# Autodesk Inventor assembly: MHPUS306-50-25-A
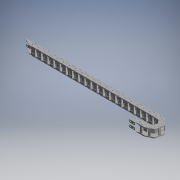
[picture p0: Inventor's stored thumbnail of the model, 180x180]
Saved by Autodesk Inventor 2017.3 (Build 213256000, 256)
## iProperties
Category: PARTsolutions
Company: MISUMI
Part Number: MHPUS306-50-25-A
Catalog Web Link: www.cadenas.de
Description: MHPUS-Cable Carriers - Flap Open-Close Type
Vendor: MISUMI
Document SubType Name: Assembly
Designer: partserver
Manufacturer: MISUMI
Mass: 772.343 g
Surface Area: 4615.68 cm^2
Volume: 772.343 cm^3
Density: 1 g/cm^3
Title: MHPUS306-50-25-A
Author: Cadenas PARTsolutions
Comments: Cable Carriers - Flap Open-Close Type
PSOL_IDENT_0: {$CADENAS_DATA\23d-libs\misumi\metric\07_slide_rails\mhpus_asmtab.prj},191 {VTYP=3D},{STYP=ASSTAB},{
PSOL_IDENT_1: NB=MHPUS306-50-25-A},{LINA=MHPUS306-50-25-A},{NN=MHPUS},{DATE=30.06.2021 12:53:59},{GEOMDATE=16.03.2
PSOL_IDENT_2: 015},{VERSION=},{LINEID=90},{WBVAR=BR,NOL,AD},{WBNUMERIC=BR,NOL}  {NB=MHPUS306-50-25-A},{LINA=MHPUS3
PSOL_IDENT_3: 06-50-25-A},{KT=DUMMY},{PN=MHPUS306-50-25-A},{MATB=Nylon 6 + Glass 20 percent},{OT=-10~80},{MATFB=Lo
PSOL_IDENT_4: w Carbon SteelC},{STFB=Trivalent Bright Chromate Plating},{NO=306},{BR=50},{BRA=50,100},{NOL=25},{NO
PSOL_IDENT_5: LALG=[6-38/1]},{AD=A},{ADALG= 'A', 'Outer circumference', 'B', 'Inner circumference' },{A=24.0},{B=3
PSOL_IDENT_6: 4},{C=44},{W=60},{P=45},{LL=60},{F=40},{T=24},{J=20},{N=7.0},{P1F=35.6},{P2F=55.6},{P1FX=32},{P2FX=5
PSOL_IDENT_7: 2},{H=134},{H1=100},{HF=160},{K=257.0},{WT=0.64},{ANGLE=53.48737},{ANGLE2=0.00000},{ANGLE3=90.00000}
PSOL_IDENT_8: ,{GAMA=27.52031},{GAMA2=0.00000},{GAMA3=nan},{BETA=45.50496},{BETA2=0.00000},{BETA3=0.00000},{X0=17.
PSOL_IDENT_9: 00000},{Y0=0.00000},{X1=-28.00000},{Y1=0.00000},{X2=-54.77500},{Y2=36.16766},{X3=-41.63725},{Y3=79.2
PSOL_IDENT_10: 0717},{X4=0.77167},{Y4=94.25653},{X5=38.10054},{Y5=69.12576},{X6=0.00000},{Y6=0.00000},{X7=0.00000},
PSOL_IDENT_11: {Y7=100.00000},{X8=45.00000},{Y8=100.00000},{R1=11.5},{R2=8.0},{R3=2.000},{L1=3.500},{L2=19.6905},{L
PSOL_IDENT_12: 3=3.700},{CL1=-26.743683950},{CL2=-53.487367900},{CL3=-53.487367900},{CL4=-42.613450190},{CL5=-3.668
PSOL_IDENT_13: 130050},{CL6=0.000000000},{CL7=0.000000000},{CL8=0.000000000},{CL9=0.000000000},{CL10=0.000000000},{
PSOL_IDENT_14: CL11=0.000000000},{CL12=0.000000000},{TILT=0},{PPATH=mhpus_asmtpl.prj}
NB: MHPUS306-50-25-A
NN: MHPUS
NT: Cable Carriers - Flap Open-Close Type
NBSYN: $PN.
LINA: MHPUS306-50-25-A
CATALOG: Misumi
PN: MHPUS306-50-25-A
MATB: Nylon 6 + Glass 20 percent
OT: -10~80
MATFB: Low Carbon SteelC
STFB: Trivalent Bright Chromate Plating
NO: 306
BR: 50
NOL: 25
AD: Outer circumference
A: 24
B: 34
C: 44
W: 60
P: 45
LL: 60
F: 40
T: 24
J: 20
N: 7
P1F: 35.6
P2F: 55.6
P1FX: 32
P2FX: 52
H: 134
H1: 100
HF: 160
K: 257
WT: 0.64
SUPPLIER: MISUMI
ARTICLENO: MHPUS306-50-25-A
BOMINFO: MHPUS306-50-25-A
CREATOR: CADENAS GmbH
## Documents named in this file (6)
- e:\temp\worker_7\temp\exporttempdir_952_134_K7orS\format_0\MHPUS306-50-25-A.iam
- e:\temp\worker_7\temp\exporttempdir_952_134_K7orS\format_0\MHPUS306-50-25-Aclip.ipt
- e:\temp\worker_7\temp\exporttempdir_952_134_K7orS\format_0\MHPUS306-Ab_free_right.ipt
- e:\temp\worker_7\temp\exporttempdir_952_134_K7orS\format_0\MHPUS306-Ab_free_left.ipt
- e:\temp\worker_7\temp\exporttempdir_952_134_K7orS\format_0\MHPUS306-Ab_fixed_right.ipt
- e:\temp\worker_7\temp\exporttempdir_952_134_K7orS\format_0\MHPUS306-Ab_fixed_left.ipt
## Components (29 placed, 5 different names)
1. MHPUS306-50-25-Aclip:1 — clip_back_to_clip_front_XY@1 <-> clip_front_to_clip_back_XY@2, clip_back_to_clip_front_Z@1 <-> clip_front_to_clip_back_Z@2, clip_front_to_fitting_fixed_right_XY@1 <-> fix_end_r_XY@28, clip_front_to_fitting_fixed_right_Z@1 <-> fix_end_r_Z@28, clip_front_to_fitting_fixed_right_YZ@1 <-> fix_end_r_YZ@28, clip_front_to_fitting_fixed_left_XY@1 <-> fix_end_l_XY@29, clip_front_to_fitting_fixed_left_Z@1 <-> fix_end_l_Z@29, clip_front_to_fitting_fixed_left_YZ@1 <-> fix_end_l_YZ@29
2. MHPUS306-50-25-Aclip:2 — clip_back_to_clip_front_XY@1 <-> clip_front_to_clip_back_XY@2, clip_back_to_clip_front_Z@1 <-> clip_front_to_clip_back_Z@2, clip_back_to_clip_front_XY@2 <-> clip_front_to_clip_back_XY@3, clip_back_to_clip_front_Z@2 <-> clip_front_to_clip_back_Z@3
3. MHPUS306-50-25-Aclip:3 — clip_back_to_clip_front_XY@2 <-> clip_front_to_clip_back_XY@3, clip_back_to_clip_front_Z@2 <-> clip_front_to_clip_back_Z@3, clip_back_to_clip_front_XY@3 <-> clip_front_to_clip_back_XY@4, clip_back_to_clip_front_Z@3 <-> clip_front_to_clip_back_Z@4
4. MHPUS306-50-25-Aclip:4 — clip_back_to_clip_front_XY@3 <-> clip_front_to_clip_back_XY@4, clip_back_to_clip_front_Z@3 <-> clip_front_to_clip_back_Z@4, clip_back_to_clip_front_XY@4 <-> clip_front_to_clip_back_XY@5, clip_back_to_clip_front_Z@4 <-> clip_front_to_clip_back_Z@5
5. MHPUS306-50-25-Aclip:5 — clip_back_to_clip_front_XY@4 <-> clip_front_to_clip_back_XY@5, clip_back_to_clip_front_Z@4 <-> clip_front_to_clip_back_Z@5, clip_back_to_clip_front_XY@5 <-> clip_front_to_clip_back_XY@6, clip_back_to_clip_front_Z@5 <-> clip_front_to_clip_back_Z@6
6. MHPUS306-50-25-Aclip:6 — clip_back_to_clip_front_XY@5 <-> clip_front_to_clip_back_XY@6, clip_back_to_clip_front_Z@5 <-> clip_front_to_clip_back_Z@6, clip_back_to_clip_front_XY@6 <-> clip_front_to_clip_back_XY@7, clip_back_to_clip_front_Z@6 <-> clip_front_to_clip_back_Z@7, clip_end_to_fitting_free_right_XY@6 <-> free_end_r_XY@26, clip_end_to_fitting_free_right_Z@6 <-> free_end_r_Z@26, clip_end_to_fitting_free_right_YZ@6 <-> free_end_r_YZ@26, clip_end_to_fitting_free_left_XY@6 <-> free_end_l_XY@27, clip_end_to_fitting_free_left_Z@6 <-> free_end_l_Z@27, clip_end_to_fitting_free_left_YZ@6 <-> free_end_l_YZ@27
7. MHPUS306-50-25-Aclip:7 — clip_back_to_clip_front_XY@6 <-> clip_front_to_clip_back_XY@7, clip_back_to_clip_front_Z@6 <-> clip_front_to_clip_back_Z@7, clip_back_to_clip_front_XY@7 <-> clip_front_to_clip_back_XY@8, clip_back_to_clip_front_Z@7 <-> clip_front_to_clip_back_Z@8
8. MHPUS306-50-25-Aclip:8 — clip_back_to_clip_front_XY@7 <-> clip_front_to_clip_back_XY@8, clip_back_to_clip_front_Z@7 <-> clip_front_to_clip_back_Z@8, clip_back_to_clip_front_XY@8 <-> clip_front_to_clip_back_XY@9, clip_back_to_clip_front_Z@8 <-> clip_front_to_clip_back_Z@9
9. MHPUS306-50-25-Aclip:9 — clip_back_to_clip_front_XY@8 <-> clip_front_to_clip_back_XY@9, clip_back_to_clip_front_Z@8 <-> clip_front_to_clip_back_Z@9, clip_back_to_clip_front_XY@9 <-> clip_front_to_clip_back_XY@10, clip_back_to_clip_front_Z@9 <-> clip_front_to_clip_back_Z@10
10. MHPUS306-50-25-Aclip:10 — clip_back_to_clip_front_XY@9 <-> clip_front_to_clip_back_XY@10, clip_back_to_clip_front_Z@9 <-> clip_front_to_clip_back_Z@10, clip_back_to_clip_front_XY@10 <-> clip_front_to_clip_back_XY@11, clip_back_to_clip_front_Z@10 <-> clip_front_to_clip_back_Z@11
11. MHPUS306-50-25-Aclip:11 — clip_back_to_clip_front_XY@10 <-> clip_front_to_clip_back_XY@11, clip_back_to_clip_front_Z@10 <-> clip_front_to_clip_back_Z@11, clip_back_to_clip_front_XY@11 <-> clip_front_to_clip_back_XY@12, clip_back_to_clip_front_Z@11 <-> clip_front_to_clip_back_Z@12
12. MHPUS306-50-25-Aclip:12 — clip_back_to_clip_front_XY@11 <-> clip_front_to_clip_back_XY@12, clip_back_to_clip_front_Z@11 <-> clip_front_to_clip_back_Z@12, clip_back_to_clip_front_XY@12 <-> clip_front_to_clip_back_XY@13, clip_back_to_clip_front_Z@12 <-> clip_front_to_clip_back_Z@13
13. MHPUS306-50-25-Aclip:13 — clip_back_to_clip_front_XY@12 <-> clip_front_to_clip_back_XY@13, clip_back_to_clip_front_Z@12 <-> clip_front_to_clip_back_Z@13, clip_back_to_clip_front_XY@13 <-> clip_front_to_clip_back_XY@14, clip_back_to_clip_front_Z@13 <-> clip_front_to_clip_back_Z@14
14. MHPUS306-50-25-Aclip:14 — clip_back_to_clip_front_XY@13 <-> clip_front_to_clip_back_XY@14, clip_back_to_clip_front_Z@13 <-> clip_front_to_clip_back_Z@14, clip_back_to_clip_front_XY@14 <-> clip_front_to_clip_back_XY@15, clip_back_to_clip_front_Z@14 <-> clip_front_to_clip_back_Z@15
15. MHPUS306-50-25-Aclip:15 — clip_back_to_clip_front_XY@14 <-> clip_front_to_clip_back_XY@15, clip_back_to_clip_front_Z@14 <-> clip_front_to_clip_back_Z@15, clip_back_to_clip_front_XY@15 <-> clip_front_to_clip_back_XY@16, clip_back_to_clip_front_Z@15 <-> clip_front_to_clip_back_Z@16
16. MHPUS306-50-25-Aclip:16 — clip_back_to_clip_front_XY@15 <-> clip_front_to_clip_back_XY@16, clip_back_to_clip_front_Z@15 <-> clip_front_to_clip_back_Z@16, clip_back_to_clip_front_XY@16 <-> clip_front_to_clip_back_XY@17, clip_back_to_clip_front_Z@16 <-> clip_front_to_clip_back_Z@17
17. MHPUS306-50-25-Aclip:17 — clip_back_to_clip_front_XY@16 <-> clip_front_to_clip_back_XY@17, clip_back_to_clip_front_Z@16 <-> clip_front_to_clip_back_Z@17, clip_back_to_clip_front_XY@17 <-> clip_front_to_clip_back_XY@18, clip_back_to_clip_front_Z@17 <-> clip_front_to_clip_back_Z@18
18. MHPUS306-50-25-Aclip:18 — clip_back_to_clip_front_XY@17 <-> clip_front_to_clip_back_XY@18, clip_back_to_clip_front_Z@17 <-> clip_front_to_clip_back_Z@18, clip_back_to_clip_front_XY@18 <-> clip_front_to_clip_back_XY@19, clip_back_to_clip_front_Z@18 <-> clip_front_to_clip_back_Z@19
19. MHPUS306-50-25-Aclip:19 — clip_back_to_clip_front_XY@18 <-> clip_front_to_clip_back_XY@19, clip_back_to_clip_front_Z@18 <-> clip_front_to_clip_back_Z@19, clip_back_to_clip_front_XY@19 <-> clip_front_to_clip_back_XY@20, clip_back_to_clip_front_Z@19 <-> clip_front_to_clip_back_Z@20
20. MHPUS306-50-25-Aclip:20 — clip_back_to_clip_front_XY@19 <-> clip_front_to_clip_back_XY@20, clip_back_to_clip_front_Z@19 <-> clip_front_to_clip_back_Z@20, clip_back_to_clip_front_XY@20 <-> clip_front_to_clip_back_XY@21, clip_back_to_clip_front_Z@20 <-> clip_front_to_clip_back_Z@21
21. MHPUS306-50-25-Aclip:21 — clip_back_to_clip_front_XY@20 <-> clip_front_to_clip_back_XY@21, clip_back_to_clip_front_Z@20 <-> clip_front_to_clip_back_Z@21, clip_back_to_clip_front_XY@21 <-> clip_front_to_clip_back_XY@22, clip_back_to_clip_front_Z@21 <-> clip_front_to_clip_back_Z@22
22. MHPUS306-50-25-Aclip:22 — clip_back_to_clip_front_XY@21 <-> clip_front_to_clip_back_XY@22, clip_back_to_clip_front_Z@21 <-> clip_front_to_clip_back_Z@22, clip_back_to_clip_front_XY@22 <-> clip_front_to_clip_back_XY@23, clip_back_to_clip_front_Z@22 <-> clip_front_to_clip_back_Z@23
23. MHPUS306-50-25-Aclip:23 — clip_back_to_clip_front_XY@22 <-> clip_front_to_clip_back_XY@23, clip_back_to_clip_front_Z@22 <-> clip_front_to_clip_back_Z@23, clip_back_to_clip_front_XY@23 <-> clip_front_to_clip_back_XY@24, clip_back_to_clip_front_Z@23 <-> clip_front_to_clip_back_Z@24
24. MHPUS306-50-25-Aclip:24 — clip_back_to_clip_front_XY@23 <-> clip_front_to_clip_back_XY@24, clip_back_to_clip_front_Z@23 <-> clip_front_to_clip_back_Z@24, clip_back_to_clip_front_XY@24 <-> clip_front_to_clip_back_XY@25, clip_back_to_clip_front_Z@24 <-> clip_front_to_clip_back_Z@25
25. MHPUS306-50-25-Aclip:25 — clip_back_to_clip_front_XY@24 <-> clip_front_to_clip_back_XY@25, clip_back_to_clip_front_Z@24 <-> clip_front_to_clip_back_Z@25
26. MHPUS306-Ab_free_right:1 — clip_end_to_fitting_free_right_XY@6 <-> free_end_r_XY@26, clip_end_to_fitting_free_right_Z@6 <-> free_end_r_Z@26, clip_end_to_fitting_free_right_YZ@6 <-> free_end_r_YZ@26
27. MHPUS306-Ab_free_left:1 — clip_end_to_fitting_free_left_XY@6 <-> free_end_l_XY@27, clip_end_to_fitting_free_left_Z@6 <-> free_end_l_Z@27, clip_end_to_fitting_free_left_YZ@6 <-> free_end_l_YZ@27
28. MHPUS306-Ab_fixed_right:1 — clip_front_to_fitting_fixed_right_XY@1 <-> fix_end_r_XY@28, clip_front_to_fitting_fixed_right_Z@1 <-> fix_end_r_Z@28, clip_front_to_fitting_fixed_right_YZ@1 <-> fix_end_r_YZ@28
29. MHPUS306-Ab_fixed_left:1 — clip_front_to_fitting_fixed_left_XY@1 <-> fix_end_l_XY@29, clip_front_to_fitting_fixed_left_Z@1 <-> fix_end_l_Z@29, clip_front_to_fitting_fixed_left_YZ@1 <-> fix_end_l_YZ@29
## Relationships (60: Mate 32, Flush 24, Angle 4)
- clip_back_to_clip_front_XY@1 <-> clip_front_to_clip_back_XY@2 [Flush]: MHPUS306-50-25-Aclip:1 ↔ MHPUS306-50-25-Aclip:2
- clip_back_to_clip_front_Z@1 <-> clip_front_to_clip_back_Z@2 [Mate]: MHPUS306-50-25-Aclip:1 ↔ MHPUS306-50-25-Aclip:2
- clip_back_to_clip_front_XY@2 <-> clip_front_to_clip_back_XY@3 [Flush]: MHPUS306-50-25-Aclip:2 ↔ MHPUS306-50-25-Aclip:3
- clip_back_to_clip_front_Z@2 <-> clip_front_to_clip_back_Z@3 [Mate]: MHPUS306-50-25-Aclip:2 ↔ MHPUS306-50-25-Aclip:3
- clip_back_to_clip_front_XY@3 <-> clip_front_to_clip_back_XY@4 [Flush]: MHPUS306-50-25-Aclip:3 ↔ MHPUS306-50-25-Aclip:4
- clip_back_to_clip_front_Z@3 <-> clip_front_to_clip_back_Z@4 [Mate]: MHPUS306-50-25-Aclip:3 ↔ MHPUS306-50-25-Aclip:4
- clip_back_to_clip_front_XY@4 <-> clip_front_to_clip_back_XY@5 [Flush]: MHPUS306-50-25-Aclip:4 ↔ MHPUS306-50-25-Aclip:5
- clip_back_to_clip_front_Z@4 <-> clip_front_to_clip_back_Z@5 [Mate]: MHPUS306-50-25-Aclip:4 ↔ MHPUS306-50-25-Aclip:5
- clip_back_to_clip_front_XY@5 <-> clip_front_to_clip_back_XY@6 [Flush]: MHPUS306-50-25-Aclip:5 ↔ MHPUS306-50-25-Aclip:6
- clip_back_to_clip_front_Z@5 <-> clip_front_to_clip_back_Z@6 [Mate]: MHPUS306-50-25-Aclip:5 ↔ MHPUS306-50-25-Aclip:6
- clip_back_to_clip_front_XY@6 <-> clip_front_to_clip_back_XY@7 [Flush]: MHPUS306-50-25-Aclip:6 ↔ MHPUS306-50-25-Aclip:7
- clip_back_to_clip_front_Z@6 <-> clip_front_to_clip_back_Z@7 [Mate]: MHPUS306-50-25-Aclip:6 ↔ MHPUS306-50-25-Aclip:7
- clip_back_to_clip_front_XY@7 <-> clip_front_to_clip_back_XY@8 [Flush]: MHPUS306-50-25-Aclip:7 ↔ MHPUS306-50-25-Aclip:8
- clip_back_to_clip_front_Z@7 <-> clip_front_to_clip_back_Z@8 [Mate]: MHPUS306-50-25-Aclip:7 ↔ MHPUS306-50-25-Aclip:8
- clip_back_to_clip_front_XY@8 <-> clip_front_to_clip_back_XY@9 [Flush]: MHPUS306-50-25-Aclip:8 ↔ MHPUS306-50-25-Aclip:9
- clip_back_to_clip_front_Z@8 <-> clip_front_to_clip_back_Z@9 [Mate]: MHPUS306-50-25-Aclip:8 ↔ MHPUS306-50-25-Aclip:9
- clip_back_to_clip_front_XY@9 <-> clip_front_to_clip_back_XY@10 [Flush]: MHPUS306-50-25-Aclip:9 ↔ MHPUS306-50-25-Aclip:10
- clip_back_to_clip_front_Z@9 <-> clip_front_to_clip_back_Z@10 [Mate]: MHPUS306-50-25-Aclip:9 ↔ MHPUS306-50-25-Aclip:10
- clip_back_to_clip_front_XY@10 <-> clip_front_to_clip_back_XY@11 [Flush]: MHPUS306-50-25-Aclip:10 ↔ MHPUS306-50-25-Aclip:11
- clip_back_to_clip_front_Z@10 <-> clip_front_to_clip_back_Z@11 [Mate]: MHPUS306-50-25-Aclip:10 ↔ MHPUS306-50-25-Aclip:11
- clip_back_to_clip_front_XY@11 <-> clip_front_to_clip_back_XY@12 [Flush]: MHPUS306-50-25-Aclip:11 ↔ MHPUS306-50-25-Aclip:12
- clip_back_to_clip_front_Z@11 <-> clip_front_to_clip_back_Z@12 [Mate]: MHPUS306-50-25-Aclip:11 ↔ MHPUS306-50-25-Aclip:12
- clip_back_to_clip_front_XY@12 <-> clip_front_to_clip_back_XY@13 [Flush]: MHPUS306-50-25-Aclip:12 ↔ MHPUS306-50-25-Aclip:13
- clip_back_to_clip_front_Z@12 <-> clip_front_to_clip_back_Z@13 [Mate]: MHPUS306-50-25-Aclip:12 ↔ MHPUS306-50-25-Aclip:13
- clip_back_to_clip_front_XY@13 <-> clip_front_to_clip_back_XY@14 [Flush]: MHPUS306-50-25-Aclip:13 ↔ MHPUS306-50-25-Aclip:14
- clip_back_to_clip_front_Z@13 <-> clip_front_to_clip_back_Z@14 [Mate]: MHPUS306-50-25-Aclip:13 ↔ MHPUS306-50-25-Aclip:14
- clip_back_to_clip_front_XY@14 <-> clip_front_to_clip_back_XY@15 [Flush]: MHPUS306-50-25-Aclip:14 ↔ MHPUS306-50-25-Aclip:15
- clip_back_to_clip_front_Z@14 <-> clip_front_to_clip_back_Z@15 [Mate]: MHPUS306-50-25-Aclip:14 ↔ MHPUS306-50-25-Aclip:15
- clip_back_to_clip_front_XY@15 <-> clip_front_to_clip_back_XY@16 [Flush]: MHPUS306-50-25-Aclip:15 ↔ MHPUS306-50-25-Aclip:16
- clip_back_to_clip_front_Z@15 <-> clip_front_to_clip_back_Z@16 [Mate]: MHPUS306-50-25-Aclip:15 ↔ MHPUS306-50-25-Aclip:16
- clip_back_to_clip_front_XY@16 <-> clip_front_to_clip_back_XY@17 [Flush]: MHPUS306-50-25-Aclip:16 ↔ MHPUS306-50-25-Aclip:17
- clip_back_to_clip_front_Z@16 <-> clip_front_to_clip_back_Z@17 [Mate]: MHPUS306-50-25-Aclip:16 ↔ MHPUS306-50-25-Aclip:17
- clip_back_to_clip_front_XY@17 <-> clip_front_to_clip_back_XY@18 [Flush]: MHPUS306-50-25-Aclip:17 ↔ MHPUS306-50-25-Aclip:18
- clip_back_to_clip_front_Z@17 <-> clip_front_to_clip_back_Z@18 [Mate]: MHPUS306-50-25-Aclip:17 ↔ MHPUS306-50-25-Aclip:18
- clip_back_to_clip_front_XY@18 <-> clip_front_to_clip_back_XY@19 [Flush]: MHPUS306-50-25-Aclip:18 ↔ MHPUS306-50-25-Aclip:19
- clip_back_to_clip_front_Z@18 <-> clip_front_to_clip_back_Z@19 [Mate]: MHPUS306-50-25-Aclip:18 ↔ MHPUS306-50-25-Aclip:19
- clip_back_to_clip_front_XY@19 <-> clip_front_to_clip_back_XY@20 [Flush]: MHPUS306-50-25-Aclip:19 ↔ MHPUS306-50-25-Aclip:20
- clip_back_to_clip_front_Z@19 <-> clip_front_to_clip_back_Z@20 [Mate]: MHPUS306-50-25-Aclip:19 ↔ MHPUS306-50-25-Aclip:20
- clip_back_to_clip_front_XY@20 <-> clip_front_to_clip_back_XY@21 [Flush]: MHPUS306-50-25-Aclip:20 ↔ MHPUS306-50-25-Aclip:21
- clip_back_to_clip_front_Z@20 <-> clip_front_to_clip_back_Z@21 [Mate]: MHPUS306-50-25-Aclip:20 ↔ MHPUS306-50-25-Aclip:21
- clip_back_to_clip_front_XY@21 <-> clip_front_to_clip_back_XY@22 [Flush]: MHPUS306-50-25-Aclip:21 ↔ MHPUS306-50-25-Aclip:22
- clip_back_to_clip_front_Z@21 <-> clip_front_to_clip_back_Z@22 [Mate]: MHPUS306-50-25-Aclip:21 ↔ MHPUS306-50-25-Aclip:22
- clip_back_to_clip_front_XY@22 <-> clip_front_to_clip_back_XY@23 [Flush]: MHPUS306-50-25-Aclip:22 ↔ MHPUS306-50-25-Aclip:23
- clip_back_to_clip_front_Z@22 <-> clip_front_to_clip_back_Z@23 [Mate]: MHPUS306-50-25-Aclip:22 ↔ MHPUS306-50-25-Aclip:23
- clip_back_to_clip_front_XY@23 <-> clip_front_to_clip_back_XY@24 [Flush]: MHPUS306-50-25-Aclip:23 ↔ MHPUS306-50-25-Aclip:24
- clip_back_to_clip_front_Z@23 <-> clip_front_to_clip_back_Z@24 [Mate]: MHPUS306-50-25-Aclip:23 ↔ MHPUS306-50-25-Aclip:24
- clip_back_to_clip_front_XY@24 <-> clip_front_to_clip_back_XY@25 [Flush]: MHPUS306-50-25-Aclip:24 ↔ MHPUS306-50-25-Aclip:25
- clip_back_to_clip_front_Z@24 <-> clip_front_to_clip_back_Z@25 [Mate]: MHPUS306-50-25-Aclip:24 ↔ MHPUS306-50-25-Aclip:25
- clip_end_to_fitting_free_right_XY@6 <-> free_end_r_XY@26 [Mate]: MHPUS306-50-25-Aclip:6 ↔ MHPUS306-Ab_free_right:1
- clip_end_to_fitting_free_right_Z@6 <-> free_end_r_Z@26 [Mate]: MHPUS306-50-25-Aclip:6 ↔ MHPUS306-Ab_free_right:1
- clip_end_to_fitting_free_right_YZ@6 <-> free_end_r_YZ@26 [Angle] (0 deg): MHPUS306-50-25-Aclip:6 ↔ MHPUS306-Ab_free_right:1
- clip_end_to_fitting_free_left_XY@6 <-> free_end_l_XY@27 [Mate]: MHPUS306-50-25-Aclip:6 ↔ MHPUS306-Ab_free_left:1
- clip_end_to_fitting_free_left_Z@6 <-> free_end_l_Z@27 [Mate]: MHPUS306-50-25-Aclip:6 ↔ MHPUS306-Ab_free_left:1
- clip_end_to_fitting_free_left_YZ@6 <-> free_end_l_YZ@27 [Angle] (0 deg): MHPUS306-50-25-Aclip:6 ↔ MHPUS306-Ab_free_left:1
- clip_front_to_fitting_fixed_right_XY@1 <-> fix_end_r_XY@28 [Mate]: MHPUS306-50-25-Aclip:1 ↔ MHPUS306-Ab_fixed_right:1
- clip_front_to_fitting_fixed_right_Z@1 <-> fix_end_r_Z@28 [Mate]: MHPUS306-50-25-Aclip:1 ↔ MHPUS306-Ab_fixed_right:1
- clip_front_to_fitting_fixed_right_YZ@1 <-> fix_end_r_YZ@28 [Angle] (180 deg): MHPUS306-50-25-Aclip:1 ↔ MHPUS306-Ab_fixed_right:1
- clip_front_to_fitting_fixed_left_XY@1 <-> fix_end_l_XY@29 [Mate]: MHPUS306-50-25-Aclip:1 ↔ MHPUS306-Ab_fixed_left:1
- clip_front_to_fitting_fixed_left_Z@1 <-> fix_end_l_Z@29 [Mate]: MHPUS306-50-25-Aclip:1 ↔ MHPUS306-Ab_fixed_left:1
- clip_front_to_fitting_fixed_left_YZ@1 <-> fix_end_l_YZ@29 [Angle] (180 deg): MHPUS306-50-25-Aclip:1 ↔ MHPUS306-Ab_fixed_left:1
